# Autodesk Inventor assembly: base_assembly
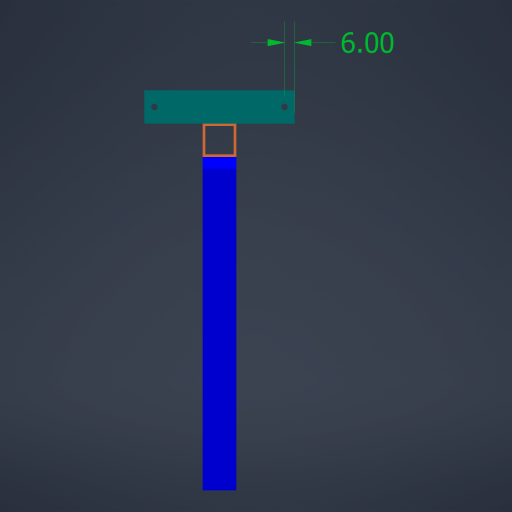
[picture p0: Inventor's stored thumbnail of the model, 512x512]
Saved by Autodesk Inventor 2024 (Build 280153000, 153)
## iProperties
Created: 2023-04-14
Part Number: base_assembly
Document SubType Name: Assembly
Designer: user
Author: user
## Documents named in this file (5)
- D:\Docs\Robot\3d\base\base_assembly.iam
- D:\Docs\Robot\3d\base\main axis.ipt
- D:\Docs\Robot\3d\base\section.ipt
- D:\Docs\Robot\3d\base\shock_absorber_holder_down_150.ipt
- D:\Docs\Robot\3d\base\shock_absorber_holder_down_200.ipt
## Components (8 placed, 4 different names)
1. main axis:1 — Совмещение:1, Совмещение:2, Плоский:1, Совмещение:48, Совмещение:50, Заподлицо:2, Заподлицо:4, Совмещение:51, Заподлицо:5, Совмещение:57, Совмещение:58
2. section:1 — Совмещение:1, Совмещение:2, Совмещение:46, Совмещение:49, Заподлицо:1, Совмещение:55, Совмещение:56
3. section:3 — Совмещение:55, Совмещение:56, Совмещение:57
4. section:4 — Совмещение:53, Совмещение:54, Совмещение:58
5. section:5 — Совмещение:45, Совмещение:47, Совмещение:48, Совмещение:49, Заподлицо:3, Совмещение:53, Совмещение:54
6. shock_absorber_holder_down_150:1 — Плоский:1, Заподлицо:3, Заподлицо:4
7. shock_absorber_holder_down_150:2 — Совмещение:50, Заподлицо:1, Заподлицо:2, Совмещение:52
8. shock_absorber_holder_down_200:1 — Совмещение:51, Совмещение:52, Заподлицо:5
## Relationships (22: Mate 16, Flush 5, PlanarJoint 1)
- Совмещение:1 [Mate]: main axis:1 ↔ section:1
- Совмещение:2 [Mate] (55 mm): main axis:1 ↔ section:1
- Плоский:1 [PlanarJoint]: main axis:1 ↔ shock_absorber_holder_down_150:1
- Совмещение:45 [Mate]: section:5
- Совмещение:46 [Mate]: section:1
- Совмещение:47 [Mate]: section:5
- Совмещение:48 [Mate]: main axis:1 ↔ section:5
- Совмещение:49 [Mate]: section:1 ↔ section:5
- Совмещение:50 [Mate]: main axis:1 ↔ shock_absorber_holder_down_150:2
- Заподлицо:1 [Flush] (56.5 mm): section:1 ↔ shock_absorber_holder_down_150:2
- Заподлицо:2 [Flush]: main axis:1 ↔ shock_absorber_holder_down_150:2
- Заподлицо:3 [Flush] (56.5 mm): section:5 ↔ shock_absorber_holder_down_150:1
- Заподлицо:4 [Flush]: main axis:1 ↔ shock_absorber_holder_down_150:1
- Совмещение:51 [Mate]: main axis:1 ↔ shock_absorber_holder_down_200:1
- Совмещение:52 [Mate] (117 mm): shock_absorber_holder_down_150:2 ↔ shock_absorber_holder_down_200:1
- Заподлицо:5 [Flush]: main axis:1 ↔ shock_absorber_holder_down_200:1
- Совмещение:53 [Mate] (105 mm): section:4 ↔ section:5
- Совмещение:54 [Mate]: section:4 ↔ section:5
- Совмещение:55 [Mate] (105 mm): section:1 ↔ section:3
- Совмещение:56 [Mate]: section:1 ↔ section:3
- Совмещение:57 [Mate]: main axis:1 ↔ section:3
- Совмещение:58 [Mate]: main axis:1 ↔ section:4
## Named parameters: hw = 1 mm, up_sh = 40 mm
